# Autodesk Inventor assembly: Racks
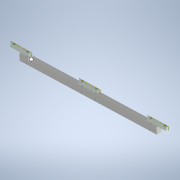
[picture p0: Inventor's stored thumbnail of the model, 180x180]
Saved by Autodesk Inventor 2022 (Build 260153000, 153)
## iProperties
Created: 2022-01-27
Part Number: Racks
Document SubType Name: Assembly
Designer: Elia
Author: Elia
## Documents named in this file (4)
- C:\Users\Elia\Documents\ELIA\UNITN\MAGISTRALE\1st year\1st semester\Mechanical Design\MDM-CyberOrto-CAD\Racks.iam
- C:\Users\Elia\Documents\ELIA\UNITN\MAGISTRALE\1st year\1st semester\Mechanical Design\MDM-CyberOrto-CAD\Rack_Pinion\Rack gear scaled1.ipt
- C:\Users\Elia\Documents\ELIA\UNITN\MAGISTRALE\1st year\1st semester\Mechanical Design\MDM-CyberOrto-CAD\Parker components\02-Fasteners\10-Standard T-Nuts\20-050.ipt
- C:\Users\Elia\Documents\ELIA\UNITN\MAGISTRALE\1st year\1st semester\Mechanical Design\MDM-CyberOrto-CAD\Parker components\02-Fasteners\16-Screws\01-Metric Screws\03-Socket Head\24-320-8SS.ipt
## Components (9 placed, 3 different names)
1. Rack gear scaled1:1 — Coincidente:1, Allineato:1, Allineato:2, Coincidente:2, Angolo:1, Allineato:4, Coincidente:6, Allineato:5, Allineato:6, Coincidente:9, Coincidente:14, Coincidente:15
2. Rack gear scaled1:2 — Coincidente:1, Allineato:1, Allineato:2, Coincidente:7, Allineato:7, Coincidente:10, Coincidente:11, Coincidente:12, Coincidente:13
3. 20-050:1 — Angolo:2, Allineato:3, Coincidente:5, Coincidente:6, Coincidente:7, Allineato:6
4. 20-050:2 — Allineato:5, Coincidente:16
5. 20-050:3 — Allineato:7, Coincidente:17
6. 24-320-8SS:1 — Coincidente:9, Coincidente:16
7. 24-320-8SS:2 — Coincidente:14, Coincidente:15
8. 24-320-8SS:3 — Coincidente:12, Coincidente:13
9. 24-320-8SS:4 — Coincidente:10, Coincidente:11, Coincidente:17
## Relationships (24: Mate 15, Flush 7, Angle 2)
- Coincidente:1 [Mate]: Rack gear scaled1:1 ↔ Rack gear scaled1:2
- Allineato:1 [Flush]: Rack gear scaled1:1 ↔ Rack gear scaled1:2
- Allineato:2 [Flush]: Rack gear scaled1:1 ↔ Rack gear scaled1:2
- Coincidente:2 [Mate]: Rack gear scaled1:1
- Angolo:1 [Angle] (90 deg): Rack gear scaled1:1
- Angolo:2 [Angle] (90 deg): 20-050:1
- Allineato:3 [Flush] (-27.5 mm): 20-050:1
- Coincidente:4 [Mate]
- Allineato:4 [Flush] (-6.4645 mm): Rack gear scaled1:1
- Coincidente:5 [Mate]: 20-050:1
- Coincidente:6 [Mate]: Rack gear scaled1:1 ↔ 20-050:1
- Coincidente:7 [Mate]: Rack gear scaled1:2 ↔ 20-050:1
- Allineato:5 [Flush] (23.224 mm): Rack gear scaled1:1 ↔ 20-050:2
- Allineato:6 [Flush] (23.224 mm): Rack gear scaled1:1 ↔ 20-050:1
- Allineato:7 [Flush] (23.224 mm): Rack gear scaled1:2 ↔ 20-050:3
- Coincidente:9 [Mate]: Rack gear scaled1:1 ↔ 24-320-8SS:1
- Coincidente:10 [Mate]: Rack gear scaled1:2 ↔ 24-320-8SS:4
- Coincidente:11 [Mate]: Rack gear scaled1:2 ↔ 24-320-8SS:4
- Coincidente:12 [Mate]: Rack gear scaled1:2 ↔ 24-320-8SS:3
- Coincidente:13 [Mate]: Rack gear scaled1:2 ↔ 24-320-8SS:3
- Coincidente:14 [Mate]: Rack gear scaled1:1 ↔ 24-320-8SS:2
- Coincidente:15 [Mate]: Rack gear scaled1:1 ↔ 24-320-8SS:2
- Coincidente:16 [Mate]: 20-050:2 ↔ 24-320-8SS:1
- Coincidente:17 [Mate]: 20-050:3 ↔ 24-320-8SS:4
